# Autodesk Inventor assembly: FTC_Field_2014-2015
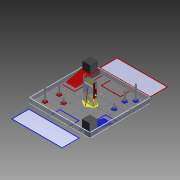
[picture p0: Inventor's stored thumbnail of the model, 180x180]
Saved by Autodesk Inventor 2015 SP1 (Build 190203100, 203)
## iProperties
Category: FTC Field Model
Company: Autodesk Inc.
Created: 2014-11-13
Part Number: FTC_Field_2014-2015
Catalog Web Link: http://www.andymark.com/FTC-Field-p/am-2970.htm
Vendor: AndyMark Inc.
Document SubType Name: Assembly
Designer: Autodesk Inc.
Author: Autodesk Inc.
## Documents named in this file (17)
- D:\Data Folder\FTC 2015\Field Model\FTC_Field_2014-2015.iam
- D:\Data Folder\FTC 2015\Field Model\Parts\Tile Field.iam
- D:\Data Folder\FTC 2015\Field Model\Parts\Center Tower 4.4r.iam
- D:\Data Folder\FTC 2015\Field Model\Parts\Pentagon Goal - 30cm.iam
- D:\Data Folder\FTC 2015\Field Model\Parts\Pentagon Goal - 90cm.iam
- D:\Data Folder\FTC 2015\Field Model\Parts\Pentagon Goal - 60cm.iam
- D:\Data Folder\FTC 2015\Field Model\Parts\FTC Field Asm.iam
- D:\Data Folder\FTC 2015\Field Model\Parts\Bucket Ramp_Red.iam
- D:\Data Folder\FTC 2015\Field Model\Parts\Bucket Ramp_Blue.iam
- D:\Data Folder\FTC 2015\Field Model\Parts\Pentagon Goal_Red- 30cm.iam
- D:\Data Folder\FTC 2015\Field Model\Parts\Pentagon Goal_Red- 60cm.iam
- D:\Data Folder\FTC 2015\Field Model\Parts\Pentagon Goal_Red - 90cm.iam
- D:\Data Folder\FTC 2015\Field Model\WiffleBall_Large.ipt
- D:\Data Folder\FTC 2015\Field Model\WiffleBall_Small.ipt
- D:\Data Folder\FTC 2015\Field Model\Simple_Robot_Starting_Size.ipt
- D:\Data Folder\FTC 2015\Field Model\Parts\Player Station_Red.ipt
- D:\Data Folder\FTC 2015\Field Model\Parts\Player Station_Blue.ipt
## Components (17 placed, 16 different names)
1. Tile Field_1 [sub-assembly] — Mate:2, Mate:5, Tangent:1, Tangent:2, Angle:1, Tangent:3, Tangent:4, Angle:2, Tangent:5, Tangent:6, Angle:3, Tangent:7, Angle:4, Tangent:8, Tangent:9, Angle:5, Tangent:10, Tangent:11, Angle:6, Mate:7, Mate:8, Mate:9, Mate:10, Mate:11, Mate:12, Mate:13, Tangent:12, Tangent:13
2. Center Tower 4.4r_2 [sub-assembly] — Mate:7, Mate:16, Angle:7
3. Bucket Ramp_Red [sub-assembly] — Mate:1, Mate:2, Mate:3, Rigid:1
4. Bucket Ramp_Blue [sub-assembly] — Mate:4, Mate:5, Mate:6, Rigid:2
5. Player Station_5
6. Player Station_6
7. Pentagon Goal - 30cm_7 [sub-assembly] — Tangent:1, Tangent:2, Angle:1
8. Pentagon Goal - 90cm_8 [sub-assembly] — Tangent:3, Tangent:4, Angle:2
9. Pentagon Goal - 60cm_9 [sub-assembly] — Tangent:5, Tangent:6, Angle:3
10. Pentagon Goal_Red - 30cm_10 [sub-assembly] — Tangent:7, Angle:4
11. Pentagon Goal_Red - 90cm_11 [sub-assembly] — Tangent:10, Tangent:11, Angle:6
12. Pentagon Goal_Red - 60cm_12 [sub-assembly] — Tangent:8, Tangent:9, Angle:5
13. FTC Field Asm_13 [sub-assembly] — Mate:1, Mate:3, Mate:4, Mate:6, Angle:7
14. WiffleBall_Large:1 — Tangent:12
15. WiffleBall_Small:1 — Tangent:13
16. Simple_Robot_Starting_Size:1 — Rigid:1
17. Simple_Robot_Starting_Size:2 — Rigid:2
## Relationships (39: Mate 17, Tangent 13, Angle 7, WeldJoint 2)
- Mate:1: Bucket Ramp_Red ↔ FTC Field Asm_13
- Mate:2: Tile Field_1 ↔ Bucket Ramp_Red
- Mate:3: Bucket Ramp_Red ↔ FTC Field Asm_13
- Mate:4: Bucket Ramp_Blue ↔ FTC Field Asm_13
- Mate:5: Tile Field_1 ↔ Bucket Ramp_Blue
- Mate:6: Bucket Ramp_Blue ↔ FTC Field Asm_13
- Tangent:1: Tile Field_1 ↔ Pentagon Goal - 30cm_7
- Tangent:2: Tile Field_1 ↔ Pentagon Goal - 30cm_7
- Angle:1 (0 deg): Tile Field_1 ↔ Pentagon Goal - 30cm_7
- Tangent:3: Tile Field_1 ↔ Pentagon Goal - 90cm_8
- Tangent:4: Tile Field_1 ↔ Pentagon Goal - 90cm_8
- Angle:2 (0 deg): Tile Field_1 ↔ Pentagon Goal - 90cm_8
- Tangent:5: Tile Field_1 ↔ Pentagon Goal - 60cm_9
- Tangent:6: Tile Field_1 ↔ Pentagon Goal - 60cm_9
- Angle:3 (0 deg): Tile Field_1 ↔ Pentagon Goal - 60cm_9
- Tangent:7: Tile Field_1 ↔ Pentagon Goal_Red - 30cm_10
- Angle:4 (0 deg): Tile Field_1 ↔ Pentagon Goal_Red - 30cm_10
- Tangent:8: Tile Field_1 ↔ Pentagon Goal_Red - 60cm_12
- Tangent:9: Tile Field_1 ↔ Pentagon Goal_Red - 60cm_12
- Angle:5 (0 deg): Tile Field_1 ↔ Pentagon Goal_Red - 60cm_12
- Tangent:10: Tile Field_1 ↔ Pentagon Goal_Red - 90cm_11
- Tangent:11: Tile Field_1 ↔ Pentagon Goal_Red - 90cm_11
- Angle:6 (0 deg): Tile Field_1 ↔ Pentagon Goal_Red - 90cm_11
- Mate:7: Tile Field_1 ↔ Center Tower 4.4r_2
- Mate:8: Tile Field_1
- Mate:9: Tile Field_1
- Mate:10: Tile Field_1
- Mate:11: Tile Field_1
- Mate:12: Tile Field_1
- Mate:13: Tile Field_1
- Mate:14
- Mate:15
- Mate:16: Center Tower 4.4r_2
- Mate:17
- Angle:7 (0 deg): Center Tower 4.4r_2 ↔ FTC Field Asm_13
- Tangent:12: Tile Field_1 ↔ WiffleBall_Large:1
- Tangent:13: Tile Field_1 ↔ WiffleBall_Small:1
- Rigid:1 [WeldJoint]: Bucket Ramp_Red ↔ Simple_Robot_Starting_Size:1
- Rigid:2 [WeldJoint]: Bucket Ramp_Blue ↔ Simple_Robot_Starting_Size:2
